# Autodesk Inventor assembly: omniwheel
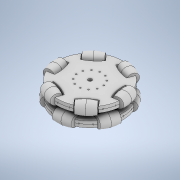
[picture p0: Inventor's stored thumbnail of the model, 180x180]
Saved by Autodesk Inventor 2021 (Build 250183000, 183)
## iProperties
Created: 2022-10-17
Part Number: omniwheel
Document SubType Name: Assembly
Designer: Jonathan
Author: Jonathan
## Documents named in this file (4)
- E:\Tron\LiDart\src\cad\omniwheel\omniwheel.iam
- E:\Tron\LiDart\src\cad\omniwheel\hub.ipt
- E:\Tron\LiDart\src\cad\omniwheel\roller_shaft.ipt
- E:\Tron\LiDart\src\cad\omniwheel\roller_half.ipt
## Components (40 placed, 3 different names)
1. hub:1 — Flush:1, Flush:2, Flush:3, Mate:3, Mate:4, Flush:4, Mate:6
2. hub:2 — Mate:3, Mate:4, Flush:4, Mate:13, Mate:15, Tangent:1, Mate:22, Tangent:2
3. hub:4 — Mate:11, Mate:13, Mate:14, Flush:6, Tangent:4
4. hub:5 — Mate:11, Mate:14, Flush:6, Mate:15, Mate:21, Tangent:3, Mate:26
5. roller_half:1 — Mate:6, Mate:23, Mate:24
6. roller_half:2 — Mate:24, Mate:25
7. roller_shaft:1 — Tangent:1, Mate:22, Tangent:2, Mate:23, Mate:25
8. roller_half:14 — Mate:21, Mate:27, Mate:28
9. roller_half:13 — Mate:28, Mate:29
10. roller_shaft:7 — Tangent:3, Mate:26, Tangent:4, Mate:27, Mate:29
11. roller_half:15
12. roller_half:16
13. roller_shaft:8
14. roller_half:25
15. roller_half:30
16. roller_shaft:13
17. roller_half:17
18. roller_half:18
19. roller_shaft:9
20. roller_half:26
21. roller_half:31
22. roller_shaft:14
23. roller_half:19
24. roller_half:20
25. roller_shaft:10
26. roller_half:27
27. roller_half:32
28. roller_shaft:15
29. roller_half:21
30. roller_half:22
31. roller_shaft:11
32. roller_half:28
33. roller_half:33
34. roller_shaft:16
35. roller_half:23
36. roller_half:24
37. roller_shaft:12
38. roller_half:29
39. roller_half:34
40. roller_shaft:17
## Component patterns: (6 elements, first: roller_half:1 + roller_half:2 + roller_shaft:1 + roller_half:14 + roller_half:13 + roller_shaft:7)
## Relationships (25: Mate 16, Flush 5, Tangent 4)
- Flush:1: hub:1
- Flush:2: hub:1
- Flush:3: hub:1
- Mate:3: hub:1 ↔ hub:2
- Mate:4: hub:1 ↔ hub:2
- Flush:4: hub:1 ↔ hub:2
- Mate:6 (1.5875 mm): hub:1 ↔ roller_half:1
- Mate:11: hub:4 ↔ hub:5
- Mate:13: hub:2 ↔ hub:4
- Mate:14: hub:4 ↔ hub:5
- Flush:6: hub:4 ↔ hub:5
- Mate:15: hub:2 ↔ hub:5
- Mate:21 (1.5875 mm): hub:5 ↔ roller_half:14
- Tangent:1: hub:2 ↔ roller_shaft:1
- Mate:22: hub:2 ↔ roller_shaft:1
- Tangent:2: hub:2 ↔ roller_shaft:1
- Mate:23: roller_half:1 ↔ roller_shaft:1
- Mate:24: roller_half:1 ↔ roller_half:2
- Mate:25: roller_half:2 ↔ roller_shaft:1
- Tangent:3: hub:5 ↔ roller_shaft:7
- Mate:26: hub:5 ↔ roller_shaft:7
- Tangent:4: hub:4 ↔ roller_shaft:7
- Mate:27: roller_half:14 ↔ roller_shaft:7
- Mate:28: roller_half:14 ↔ roller_half:13
- Mate:29: roller_half:13 ↔ roller_shaft:7
## Named parameters: roller_angle = 40 deg, wheel_d = 152.4 mm, roller_d = 25.4 mm, roller_shaft_d = 3.175 mm, roller_count = 6, hub_d = 139.7 mm, shaft_d = 8 mm, hub_t = 6.35 mm, roller_side_gap = 1.5875 mm, roller_back_gap = 1.5875 mm, roller_shaft_l = 50.8 mm
